# Autodesk Inventor assembly: WormGearExample
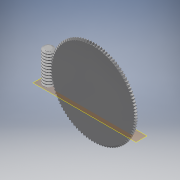
[picture p0: Inventor's stored thumbnail of the model, 180x180]
Saved by Autodesk Inventor 2019.2 (Build 232265000, 265)
## iProperties
Created: 2018-12-29
Part Number: WormGearExample
Document SubType Name: Assembly
Designer: steele
Author: steele
## Documents named in this file (2)
- C:\git\CAD-Development\robSteele\ShapeWays\WormGearExample.iam
- C:\git\CAD-Development\robSteele\ShapeWays\WormGearExample\Design Accelerator\Worm Gears2.iam
## Components (1 placed, 1 different names)
1. Worm Gears:1 [sub-assembly] — Angle:1
## Relationships (1: Angle 1)
- Angle:1 (0 deg): Worm Gears:1
